# Autodesk Inventor assembly: motorchassisholder2Ass
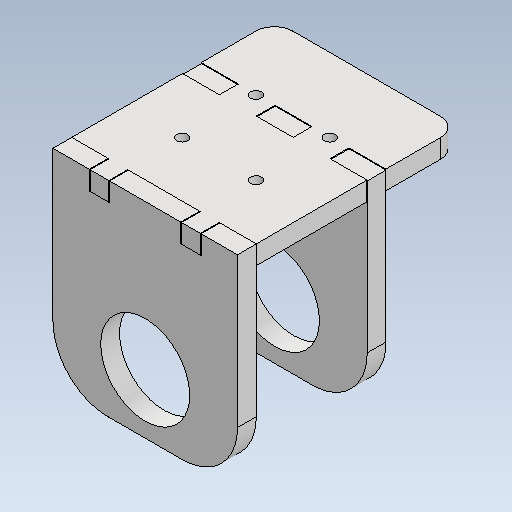
[picture p0: Inventor's stored thumbnail of the model, 512x512]
Saved by Autodesk Inventor 2025 (Build 290162000, 162)
## iProperties
Created: 2024-08-15
Part Number: motorchassisholder2Ass
Document SubType Name: Assembly
Designer: PC
Author: PC
## Documents named in this file (4)
- C:\Users\HP\Downloads\Compressed\KNIGHTS mobile platform CAD files\motorchassisholder2Ass.iam
- C:\Users\HP\Downloads\Compressed\KNIGHTS mobile platform CAD files\motor chasis holder.ipt
- C:\Users\HP\Downloads\Compressed\KNIGHTS mobile platform CAD files\motorholder1A.ipt
- C:\Users\HP\Downloads\Compressed\KNIGHTS mobile platform CAD files\inner motorholder1A.ipt
## Components (3 placed, 3 different names)
1. motor chasis holder:1 — Flush:1, Flush:2, Mate:1, Mate:2, Mate:3, Mate:4
2. motorholder1A:1 — Flush:1, Flush:2, Mate:1
3. inner motorholder1A:1 — Mate:2, Mate:3, Mate:4
## Relationships (6: Mate 4, Flush 2)
- Flush:1: motor chasis holder:1 ↔ motorholder1A:1
- Flush:2: motor chasis holder:1 ↔ motorholder1A:1
- Mate:1: motor chasis holder:1 ↔ motorholder1A:1
- Mate:2: motor chasis holder:1 ↔ inner motorholder1A:1
- Mate:3: motor chasis holder:1 ↔ inner motorholder1A:1
- Mate:4: motor chasis holder:1 ↔ inner motorholder1A:1
